# Autodesk Inventor assembly: Multi-Cat-family
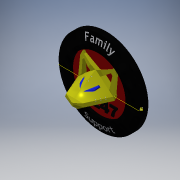
[picture p0: Inventor's stored thumbnail of the model, 180x180]
Saved by Autodesk Inventor 2016 (Build 200138000, 138)
## iProperties
Created: 2015-06-02
Part Number: Multi-Cat-family
Document SubType Name: Assembly
Designer: Spooner
Author: Spooner
## Documents named in this file (8)
- C:\Users\Spooner\Documents\Inventor\2016 RoboCat\Multi-Cat-family.iam
- C:\Users\Spooner\Documents\Inventor\2016 RoboCat\Background.ipt
- C:\Users\Spooner\Documents\Inventor\2016 RoboCat\Disk.ipt
- C:\Users\Spooner\Documents\Inventor\2016 RoboCat\Numbers.ipt
- C:\Users\Spooner\Documents\Inventor\2016 RoboCat\Cat.ipt
- C:\Users\Spooner\Documents\Inventor\2016 RoboCat\Eyes.ipt
- C:\Users\Spooner\Documents\Inventor\2016 RoboCat\Team Pin Family.ipt
- C:\Users\Spooner\Documents\Inventor\2016 RoboCat\Team Pin Family-Text.ipt
## Components (7 placed, 7 different names)
1. Background:1 — Insert:1, Angle:2, Mate:3, Mate:4, Mate:5, Mate:6
2. Disk:1 — Mate:1, Mate:2, Insert:1, Angle:1, Angle:2, Tangent:1, Angle:3, Insert:2, Angle:4
3. Numbers:1 — Mate:3, Mate:4, Mate:5
4. Cat:1 — Mate:6, Tangent:1, Angle:3, Mate:7, Mate:8, Mate:9
5. Eyes:1 — Mate:7, Mate:8, Mate:9
6. Team Pin Family:1 — Insert:2, Angle:4, Mate:10, Mate:11, Mate:12
7. Team Pin Family-Text:1 — Mate:10, Mate:11, Mate:12
## Relationships (19: Mate 12, Angle 4, Insert 2, Tangent 1)
- Mate:1: Disk:1
- Mate:2: Disk:1
- Insert:1: Background:1 ↔ Disk:1
- Angle:1 (0 deg): Disk:1
- Angle:2 (0 deg): Background:1 ↔ Disk:1
- Mate:3: Background:1 ↔ Numbers:1
- Mate:4: Background:1 ↔ Numbers:1
- Mate:5: Background:1 ↔ Numbers:1
- Mate:6: Background:1 ↔ Cat:1
- Tangent:1: Disk:1 ↔ Cat:1
- Angle:3 (0 deg): Disk:1 ↔ Cat:1
- Mate:7: Cat:1 ↔ Eyes:1
- Mate:8: Cat:1 ↔ Eyes:1
- Mate:9: Cat:1 ↔ Eyes:1
- Insert:2: Disk:1 ↔ Team Pin Family:1
- Angle:4 (0 deg): Disk:1 ↔ Team Pin Family:1
- Mate:10: Team Pin Family:1 ↔ Team Pin Family-Text:1
- Mate:11: Team Pin Family:1 ↔ Team Pin Family-Text:1
- Mate:12: Team Pin Family:1 ↔ Team Pin Family-Text:1
